# Autodesk Inventor assembly: Assembly4
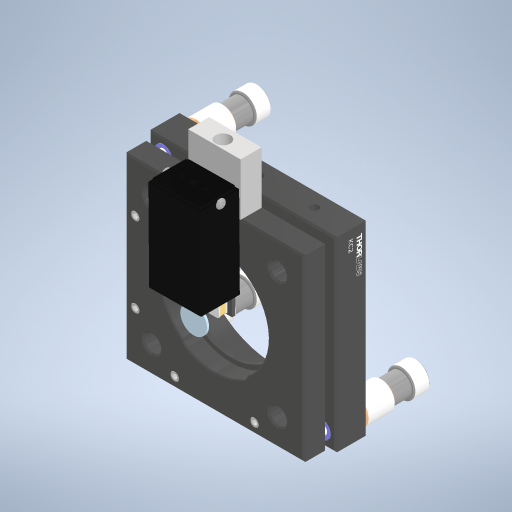
[picture p0: Inventor's stored thumbnail of the model, 512x512]
Saved by Autodesk Inventor 2023 (Build 270158000, 158)
## iProperties
Created: 2024-01-12
Part Number: Assembly4
Document SubType Name: Assembly
Designer: kerlin
Author: kerlin
## Documents named in this file (4)
- C:\Users\kerlin\Documents\KerlinLab\KTN\Multipass\MechanicalDrawing\Assembly4.iam
- C:\Users\kerlin\Downloads\KC2-Solidworks.ipt
- C:\Users\kerlin\Downloads\sc30.ipt
- C:\Users\kerlin\Documents\KerlinLab\KTN\Multipass\MechanicalDrawing\ResonantAdapter.ipt
## Components (3 placed, 3 different names)
1. KC2-Solidworks:1 — Mate:1, Mate:2, Mate:3, Mate:4
2. sc30:1 — Mate:1, Mate:2
3. ResonantAdapter:1 — Mate:3, Mate:4
## Relationships (4: Mate 4)
- Mate:1: KC2-Solidworks:1 ↔ sc30:1
- Mate:2: KC2-Solidworks:1 ↔ sc30:1
- Mate:3: KC2-Solidworks:1 ↔ ResonantAdapter:1
- Mate:4: KC2-Solidworks:1 ↔ ResonantAdapter:1
